# Autodesk Inventor assembly: 6_Omni-Directional_Wheel_217-2585
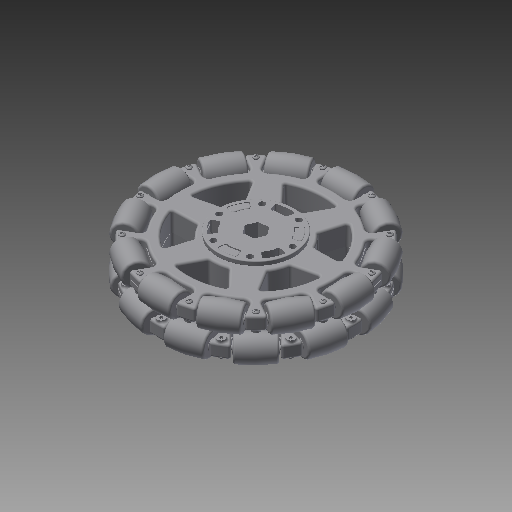
[picture p0: Inventor's stored thumbnail of the model, 512x512]
Saved by Autodesk Inventor 2018 (Build 220112000, 112)
## iProperties
Company: Microsoft
Created: 2012-12-03
Part Number: 6_Omni-Directional_Wheel_217-2585
Description: STEP AP203
Document SubType Name: Assembly
Designer: user
Mass: 335.548 g
Surface Area: 1925.33 cm^2
Volume: 335.548 cm^3
Density: 1 g/cm^3
Sending System: SolidWorks 2012
Preprocessor: SwSTEP 2.0
Title: 217-2585.20121203.STEP
Author: svradm
Revision Number: ANY
## Documents named in this file (9)
- C:\Users\user\Documents\GrabCAD\New folder\Build season\OMNIWHEEL STEP\6_Omni-Directional_Wheel_217-2585.iam
- C:\Users\user\Documents\GrabCAD\New folder\Build season\OMNIWHEEL STEP\217-2585-001 Rev1.ipt
- C:\Users\user\Documents\GrabCAD\New folder\Build season\OMNIWHEEL STEP\217-2585-002 Rev1.ipt
- C:\Users\user\Documents\GrabCAD\New folder\Build season\OMNIWHEEL STEP\217-2585-003 Rev2.ipt
- C:\Users\user\Documents\GrabCAD\New folder\Build season\OMNIWHEEL STEP\217-2585-004 Rev1.ipt
- C:\Users\user\Documents\GrabCAD\New folder\Build season\OMNIWHEEL STEP\BEAM-0750.ipt
- C:\Users\user\Documents\GrabCAD\New folder\Build season\OMNIWHEEL STEP\90116A020_90116A020.ipt
- C:\Users\user\Documents\GrabCAD\New folder\Build season\OMNIWHEEL STEP\217-2584-005 Rev1 A.ipt
- C:\Users\user\Documents\GrabCAD\New folder\Build season\OMNIWHEEL STEP\1_2_Hex_Bore_Aluminum_VersaHub_217-2592.ipt
## Components (131 placed, 130 different names)
1. 217-2585-001 Rev1_1
2. 217-2585-002 Rev1_2
3. 217-2585-001 Rev1_3
4. 217-2585-001 Rev1_4
5. 217-2585-001 Rev1_5
6. 217-2585-001 Rev1_6
7. 217-2585-001 Rev1_7
8. 217-2585-001 Rev1_8
9. 217-2585-001 Rev1_9
10. 217-2585-001 Rev1_10
11. 217-2585-001 Rev1_11
12. 217-2585-001 Rev1_12
13. 217-2585-001 Rev1_13
14. 217-2585-001 Rev1_14
15. 217-2585-003 Rev2_15 — Insert:2, Mate:1
16. 217-2585-004 Rev1_16
17. 217-2585-004 Rev1_17
18. 217-2585-003 Rev2_18 — Insert:1, Mate:2
19. 217-2585-004 Rev1_19
20. 217-2585-004 Rev1_20
21. 217-2585-004 Rev1_21
22. 217-2585-004 Rev1_22
23. 217-2585-004 Rev1_23
24. 217-2585-004 Rev1_24
25. 217-2585-004 Rev1_25
26. 217-2585-004 Rev1_26
27. 217-2585-004 Rev1_27
28. 217-2585-004 Rev1_28
29. 217-2585-004 Rev1_29
30. 217-2585-004 Rev1_30
31. 217-2585-004 Rev1_31
32. 217-2585-004 Rev1_32
33. 217-2585-004 Rev1_33
34. 217-2585-004 Rev1_34
35. 217-2585-004 Rev1_35
36. 217-2585-004 Rev1_36
37. 217-2585-004 Rev1_37
38. 217-2585-004 Rev1_38
39. 217-2585-004 Rev1_39
40. 217-2585-004 Rev1_40
41. 217-2585-001 Rev1_41
42. 217-2585-001 Rev1_42
43. 217-2585-001 Rev1_43
44. 217-2585-001 Rev1_44
45. 217-2585-001 Rev1_45
46. 217-2585-001 Rev1_46
47. 217-2585-001 Rev1_47
48. 217-2585-001 Rev1_48
49. 217-2585-001 Rev1_49
50. 217-2585-001 Rev1_50
51. 217-2585-001 Rev1_51
52. BEAM-0750_52
53. BEAM-0750_53
54. BEAM-0750_54
55. BEAM-0750_55
56. BEAM-0750_56
57. BEAM-0750_57
58. 90116A020_90116A020_58
59. 90116A020_90116A020_59
60. 90116A020_90116A020_60
61. 90116A020_90116A020_61
62. 90116A020_90116A020_62
63. 90116A020_90116A020_63
64. 90116A020_90116A020_64
65. 90116A020_90116A020_65
66. 90116A020_90116A020_66
67. 90116A020_90116A020_67
68. 90116A020_90116A020_68
69. 90116A020_90116A020_69
70. 90116A020_90116A020_70
71. 90116A020_90116A020_71
72. 90116A020_90116A020_72
73. 90116A020_90116A020_73
74. 90116A020_90116A020_74
75. 90116A020_90116A020_75
76. 90116A020_90116A020_76
77. 90116A020_90116A020_77
78. 90116A020_90116A020_78
79. 90116A020_90116A020_79
80. 90116A020_90116A020_80
81. 90116A020_90116A020_81
82. 217-2584-005 Rev1 A_82
83. 217-2584-005 Rev1 A_83
84. 217-2584-005 Rev1 A_84
85. 217-2584-005 Rev1 A_85
86. 217-2584-005 Rev1 A_86
87. 217-2584-005 Rev1 A_87
88. 217-2584-005 Rev1 A_88
89. 217-2584-005 Rev1 A_89
90. 217-2584-005 Rev1 A_90
91. 217-2584-005 Rev1 A_91
92. 217-2584-005 Rev1 A_92
93. 217-2584-005 Rev1 A_93
94. 217-2584-005 Rev1 A_94
95. 217-2584-005 Rev1 A_95
96. 217-2584-005 Rev1 A_96
97. 217-2584-005 Rev1 A_97
98. 217-2584-005 Rev1 A_98
99. 217-2584-005 Rev1 A_99
100. 217-2584-005 Rev1 A_100
101. 217-2584-005 Rev1 A_101
102. 217-2584-005 Rev1 A_102
103. 217-2584-005 Rev1 A_103
104. 217-2584-005 Rev1 A_104
105. 217-2584-005 Rev1 A_105
106. 217-2584-005 Rev1 A_106
107. 217-2584-005 Rev1 A_107
108. 217-2584-005 Rev1 A_108
109. 217-2584-005 Rev1 A_109
110. 217-2584-005 Rev1 A_110
111. 217-2584-005 Rev1 A_111
112. 217-2584-005 Rev1 A_112
113. 217-2584-005 Rev1 A_113
114. 217-2584-005 Rev1 A_114
115. 217-2584-005 Rev1 A_115
116. 217-2584-005 Rev1 A_116
117. 217-2584-005 Rev1 A_117
118. 217-2584-005 Rev1 A_118
119. 217-2584-005 Rev1 A_119
120. 217-2584-005 Rev1 A_120
121. 217-2584-005 Rev1 A_121
122. 217-2584-005 Rev1 A_122
123. 217-2584-005 Rev1 A_123
124. 217-2584-005 Rev1 A_124
125. 217-2584-005 Rev1 A_125
126. 217-2584-005 Rev1 A_126
127. 217-2584-005 Rev1 A_127
128. 217-2584-005 Rev1 A_128
129. 217-2584-005 Rev1 A_129
130. 1_2_Hex_Bore_Aluminum_VersaHub_217-2592:1 — Insert:2, Mate:1
131. 1_2_Hex_Bore_Aluminum_VersaHub_217-2592:2 — Insert:1, Mate:2
## Relationships (4: Insert 2, Mate 2)
- Insert:1: 217-2585-003 Rev2_18 ↔ 1_2_Hex_Bore_Aluminum_VersaHub_217-2592:2
- Insert:2: 217-2585-003 Rev2_15 ↔ 1_2_Hex_Bore_Aluminum_VersaHub_217-2592:1
- Mate:1: 217-2585-003 Rev2_15 ↔ 1_2_Hex_Bore_Aluminum_VersaHub_217-2592:1
- Mate:2: 217-2585-003 Rev2_18 ↔ 1_2_Hex_Bore_Aluminum_VersaHub_217-2592:2
